# Autodesk Inventor assembly: Assembled Horns
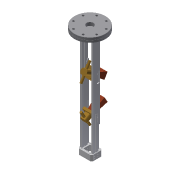
[picture p0: Inventor's stored thumbnail of the model, 180x180]
Saved by Autodesk Inventor 2015 SP1 (Build 190203100, 203)
## iProperties
Created: 2016-04-14
Part Number: Assembled Horns
Document SubType Name: Assembly
Designer: jad211
Author: jad211
## Documents named in this file (3)
- C:\ColdMatter\CADFiles\EDM Machine\Detection Region\Microwave Horn Assembly\Assembled Horns.iam
- C:\ColdMatter\CADFiles\EDM Machine\Detection Region\Microwave Horn Assembly\innerHorn slider.iam
- C:\ColdMatter\CADFiles\EDM Machine\Detection Region\Microwave Horn Assembly\outerHorn slider.iam
## Components (2 placed, 2 different names)
1. innerHorn slider:1 [sub-assembly] — Mate:1, Mate:2
2. outerHorn slider:1 [sub-assembly] — Mate:1, Mate:2
## Relationships (2: Mate 2)
- Mate:1: innerHorn slider:1 ↔ outerHorn slider:1
- Mate:2: innerHorn slider:1 ↔ outerHorn slider:1
